# Autodesk Inventor assembly: Assembly1
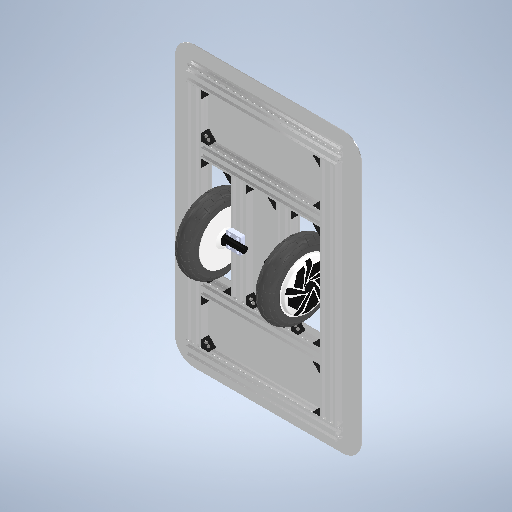
[picture p0: Inventor's stored thumbnail of the model, 512x512]
Saved by Autodesk Inventor 2025 (Build 290162000, 162)
## iProperties
Created: 2025-09-29
Part Number: Assembly1
Document SubType Name: Weldment
Designer: hp
Mass: 4352.41 g
Surface Area: 16168.4 cm^2
Volume: 1611.69 cm^3
Density: 2.70052 g/cm^3
Weld Material: Aluminum 6061, Welded
Author: hp
## Documents named in this file (16)
- D:\gp amr\Assembly1.iam
- D:\gp amr\aluminum-extrusion-beams-1.snapshot.4\2040 - V-Slot\2040 - V-Slot.ipt
- D:\gp amr\corner-brackets-2.snapshot.2\OB-Bracket 2020\OB-Bracket 2020.ipt
- D:\gp amr\nut-m4-2020-10-6mm-1.snapshot.6\2040 - V-Slot.ipt 60.ipt
- D:\gp amr\aluminum-extrusion-beams-1.snapshot.4\2040 - V-Slot\2040 - V-Slot.ipt 320.ipt
- D:\gp amr\plate2mm.ipt
- D:\gp amr\hoverboard-wheel-8-bldc-motor-1.snapshot.4\Motor, BLDC, Hoverboard Wheel, 8.0in\Motor, BLDC, Hoverboard Wheel, 8.0in.ipt
- D:\gp amr\aluminum-extrusion-beams-1.snapshot.4\2040 - V-Slot\2040 - V-Slot.ipt 280.ipt
- D:\gp amr\hoverboard-motor-shaft-retention-bracket-1.snapshot.6\Hub Motor Shaft Bracket\Hub Motor Shaft Bracket.ipt
- D:\t-nut-m5-2020s-1.snapshot.4\T NUT M5 2020S.ipt
- C:\Users\hp\OneDrive - Faculty of Engineering Ain Shams University\Documents\Inventor\Content Center Files\R2025\en-US\ISO 4762(2)\ISO 4762 - M4 x 8ISO.ipt
- D:\gp amr\Assembly1\AIP\FEA\f78c4d0io.fins
- D:\gp amr\Assembly1\AIP\FEA\f78c4d0io.fsat
- D:\gp amr\Assembly1\AIP\FEA\f78c4d0io.ftes
- D:\gp amr\Assembly1\AIP\FEA\f78c4d0io.fwiz
- D:\gp amr\Assembly1\AIP\FEA\f78c4d0ow.fmsh
## Components (114 placed, 10 different names)
1. 2040 - V-Slot:1 — Mate:4, Flush:2, Mate:7, Mate:8, Flush:3, Mate:9, Flush:4, Mate:15, Angle:5, Flush:20, Mate:42, Angle:7, Angle:8
2. 2040 - V-Slot:4 — Mate:11, Mate:12, Flush:5, Mate:17, Mate:19, Mate:21, Angle:11, Angle:12
3. OB-Bracket 2020:1 — Mate:4, Flush:2, Mate:41, Insert:1, Insert:3, Insert:46, Insert:49
4. OB-Bracket 2020:2 — Mate:15, Mate:16, Flush:8, Insert:2, Insert:4, Insert:47, Insert:48
5. OB-Bracket 2020:3 — Mate:19, Mate:20, Flush:10, Insert:7, Insert:8, Insert:54, Insert:55
6. OB-Bracket 2020:4 — Mate:31, Mate:32, Flush:15, Insert:26, Insert:27, Insert:66, Insert:67
7. OB-Bracket 2020:5 — Mate:17, Mate:18, Flush:9, Insert:5, Insert:6, Insert:56, Insert:57
8. OB-Bracket 2020:6 — Mate:23, Mate:24, Flush:11, Insert:28, Insert:29, Insert:72, Insert:73
9. OB-Bracket 2020:7 — Mate:25, Mate:26, Flush:12, Insert:18, Insert:19, Insert:50, Insert:51
10. 2040 - V-Slot.ipt 60:1 — Mate:7, Mate:8, Flush:3, Mate:13, Angle:2, Flush:6, Mate:14, Angle:3, Flush:7, Mate:18, Flush:9, Mate:28, Flush:13, Mate:30, Flush:14, Mate:36, Mate:37, Mate:41, Mate:44, Angle:10, Angle:15, Angle:21, Angle:23
11. 2040 - V-Slot.ipt 60:2 — Mate:9, Flush:4, Mate:11, Mate:12, Flush:5, Mate:16, Flush:8, Mate:20, Flush:10, Mate:24, Mate:26, Mate:32, Flush:15, Mate:34, Flush:16, Mate:39, Angle:4, Flush:19, Mate:40, Mate:47, Angle:9, Angle:17, Angle:18, Angle:25
12. 2040 - V-Slot.ipt 320:1 — Mate:13, Angle:2, Flush:6, Mate:22, Mate:25, Flush:12, Mate:29, Mate:31, Mate:35, Flush:17, Mate:39, Mate:42, Mate:45, Mate:48, Mate:56, Mate:57, Angle:14, Angle:16, Angle:22, Angle:24, Mate:68, Mate:70, Mate:73, Mate:75, Angle:34, Angle:37, Angle:39, Angle:40
13. 2040 - V-Slot.ipt 320:2 — Mate:14, Angle:3, Flush:7, Mate:21, Mate:22, Mate:23, Flush:11, Mate:27, Mate:33, Mate:38, Flush:18, Angle:13, Angle:19, Angle:20, Mate:65, Flush:25, Mate:67, Flush:26, Mate:77, Flush:32, Mate:79, Angle:26, Angle:28, Angle:31, Angle:33, Insert:76
14. OB-Bracket 2020:8 — Mate:27, Mate:28, Flush:13, Insert:22, Insert:23, Insert:74, Insert:75
15. OB-Bracket 2020:9 — Mate:29, Mate:30, Flush:14, Insert:20, Insert:21, Insert:52, Insert:53
16. OB-Bracket 2020:10 — Mate:33, Mate:34, Flush:16, Insert:16, Insert:17, Insert:58, Insert:59
17. OB-Bracket 2020:11 — Mate:35, Mate:36, Flush:17, Insert:24, Insert:25, Insert:83, Insert:84
18. OB-Bracket 2020:12 — Mate:37, Mate:38, Flush:18, Insert:14, Insert:15, Insert:60, Insert:61
19. plate2mm:1 — Angle:4, Angle:5, Flush:19, Mate:40, Flush:20, Flush:21, Flush:22, Mate:43, Mate:46
20. Motor, BLDC, Hoverboard Wheel, 8.0in:1 — Mate:61, Mate:62, Mate:63
21. Motor, BLDC, Hoverboard Wheel, 8.0in:2 — Mate:58, Mate:59, Mate:60
22. 2040 - V-Slot.ipt 280:1 — Mate:43, Mate:44, Mate:45, Mate:55, Flush:24, Mate:66, Mate:69, Flush:28, Mate:74, Flush:31, Mate:78, Flush:33, Angle:27, Angle:30, Angle:36, Angle:41
23. 2040 - V-Slot.ipt 280:2 — Mate:46, Mate:47, Mate:48, Mate:54, Flush:23, Mate:64, Mate:71, Flush:29, Mate:72, Flush:30, Mate:76, Angle:29, Angle:32, Angle:35, Angle:38
24. Hub Motor Shaft Bracket:1 — Mate:54, Mate:56, Flush:23, Mate:61, Mate:62, Mate:63
25. Hub Motor Shaft Bracket:2 — Mate:55, Mate:57, Flush:24, Mate:58, Mate:59, Mate:60
26. T NUT M5 2020S:1 — Insert:2, Angle:8
27. T NUT M5 2020S:2 — Insert:3, Angle:10
28. T NUT M5 2020S:3 — Angle:9, Insert:4
29. T NUT M5 2020S:4 — Insert:1, Angle:7
30. T NUT M5 2020S:5 — Insert:8
31. T NUT M5 2020S:6 — Insert:6, Angle:11
32. T NUT M5 2020S:7 — Insert:7, Angle:12
33. T NUT M5 2020S:8 — Insert:5
34. T NUT M5 2020S:9 — Insert:14
35. T NUT M5 2020S:10 — Insert:15
36. T NUT M5 2020S:11 — Insert:17, Angle:13
37. T NUT M5 2020S:12 — Insert:16
38. T NUT M5 2020S:13 — Insert:18, Angle:17
39. T NUT M5 2020S:14 — Insert:20, Angle:15
40. T NUT M5 2020S:15 — Insert:21, Angle:14
41. T NUT M5 2020S:16 — Insert:19, Angle:16
42. T NUT M5 2020S:17 — Insert:23, Angle:20
43. T NUT M5 2020S:18 — Insert:25, Angle:22
44. T NUT M5 2020S:19 — Insert:26, Angle:24
45. T NUT M5 2020S:20 — Insert:22, Angle:21
46. T NUT M5 2020S:21 — Insert:24, Angle:23
47. T NUT M5 2020S:22 — Insert:27, Angle:25
48. T NUT M5 2020S:23 — Insert:29, Angle:18
49. T NUT M5 2020S:24 — Insert:28, Angle:19
50. OB-Bracket 2020:13 — Mate:74, Mate:75, Flush:31, Insert:30, Insert:31, Insert:79, Insert:80
51. OB-Bracket 2020:14 — Mate:76, Mate:77, Flush:32, Insert:40, Insert:41, Insert:85, Insert:86
52. OB-Bracket 2020:15 — Mate:66, Mate:67, Flush:26, Insert:44, Insert:45, Insert:68, Insert:69
53. OB-Bracket 2020:16 — Mate:68, Mate:69, Flush:28, Insert:36, Insert:37, Insert:62, Insert:63
54. OB-Bracket 2020:17 — Mate:70, Mate:71, Flush:29, Insert:34, Insert:35, Insert:64, Insert:65
55. OB-Bracket 2020:18 — Mate:72, Mate:73, Flush:30, Insert:32, Insert:33, Insert:81, Insert:82
56. OB-Bracket 2020:19 — Mate:78, Mate:79, Flush:33, Insert:38, Insert:39, Insert:77, Insert:78
57. OB-Bracket 2020:20 — Mate:64, Mate:65, Flush:25, Insert:42, Insert:43, Insert:70, Insert:71
58. T NUT M5 2020S:25 — Insert:34, Angle:38
59. T NUT M5 2020S:26 — Insert:37, Angle:40
60. T NUT M5 2020S:27 — Insert:32, Angle:35
61. T NUT M5 2020S:28 — Insert:31, Angle:37
62. T NUT M5 2020S:29 — Insert:33, Angle:34
63. T NUT M5 2020S:30 — Insert:35, Angle:39
64. T NUT M5 2020S:31 — Insert:36, Angle:41
65. T NUT M5 2020S:32 — Insert:30, Angle:36
66. T NUT M5 2020S:33 — Insert:40, Angle:32
67. T NUT M5 2020S:34 — Insert:42, Angle:29
68. T NUT M5 2020S:35 — Insert:38, Angle:30
69. T NUT M5 2020S:36 — Insert:39, Angle:31
70. T NUT M5 2020S:37 — Insert:44, Angle:26
71. T NUT M5 2020S:38 — Insert:43, Angle:28
72. T NUT M5 2020S:39 — Insert:45, Angle:27
73. T NUT M5 2020S:40 — Insert:41, Angle:33
74. ISO 4762 M4 x 8:1 — Insert:46
75. ISO 4762 M4 x 8:2 — Insert:48
76. ISO 4762 M4 x 8:3 — Insert:51
77. ISO 4762 M4 x 8:4 — Insert:52
78. ISO 4762 M4 x 8:5 — Insert:53
79. ISO 4762 M4 x 8:6 — Insert:54
80. ISO 4762 M4 x 8:7 — Insert:55
81. ISO 4762 M4 x 8:8 — Insert:56
82. ISO 4762 M4 x 8:9 — Insert:57
83. ISO 4762 M4 x 8:10 — Insert:58
84. ISO 4762 M4 x 8:11 — Insert:61
85. ISO 4762 M4 x 8:12 — Insert:60
86. ISO 4762 M4 x 8:13 — Insert:59
87. ISO 4762 M4 x 8:14 — Insert:50
88. ISO 4762 M4 x 8:15 — Insert:49
89. ISO 4762 M4 x 8:16 — Insert:47
90. ISO 4762 M4 x 8:17 — Insert:72
91. ISO 4762 M4 x 8:18 — Insert:70
92. ISO 4762 M4 x 8:19 — Insert:71
93. ISO 4762 M4 x 8:20 — Insert:73
94. ISO 4762 M4 x 8:21 — Insert:69
95. ISO 4762 M4 x 8:22 — Insert:67
96. ISO 4762 M4 x 8:23 — Insert:74
97. ISO 4762 M4 x 8:24 — Insert:68
98. ISO 4762 M4 x 8:25 — Insert:62
99. ISO 4762 M4 x 8:26 — Insert:64
100. ISO 4762 M4 x 8:27 — Insert:75
101. ISO 4762 M4 x 8:28 — Insert:66
102. ISO 4762 M4 x 8:29 — Insert:77
103. ISO 4762 M4 x 8:30 — Insert:76
104. ISO 4762 M4 x 8:31 — Insert:65
105. ISO 4762 M4 x 8:32 — Insert:63
106. ISO 4762 M4 x 8:33 — Insert:80
107. ISO 4762 M4 x 8:34 — Insert:84
108. ISO 4762 M4 x 8:35 — Insert:83
109. ISO 4762 M4 x 8:36 — Insert:82
110. ISO 4762 M4 x 8:37 — Insert:81
111. ISO 4762 M4 x 8:38 — Insert:79
112. ISO 4762 M4 x 8:39 — Insert:78
113. ISO 4762 M4 x 8:40 — Insert:85
114. ISO 4762 M4 x 8:43 — Insert:86
## Relationships (219: Insert 81, Mate 68, Angle 39, Flush 31)
- Mate:4: 2040 - V-Slot:1 ↔ OB-Bracket 2020:1
- Flush:2: 2040 - V-Slot:1 ↔ OB-Bracket 2020:1
- Mate:7: 2040 - V-Slot:1 ↔ 2040 - V-Slot.ipt 60:1
- Mate:8: 2040 - V-Slot:1 ↔ 2040 - V-Slot.ipt 60:1
- Flush:3: 2040 - V-Slot:1 ↔ 2040 - V-Slot.ipt 60:1
- Mate:9: 2040 - V-Slot:1 ↔ 2040 - V-Slot.ipt 60:2
- Flush:4: 2040 - V-Slot:1 ↔ 2040 - V-Slot.ipt 60:2
- Mate:11: 2040 - V-Slot:4 ↔ 2040 - V-Slot.ipt 60:2
- Mate:12: 2040 - V-Slot:4 ↔ 2040 - V-Slot.ipt 60:2
- Flush:5: 2040 - V-Slot:4 ↔ 2040 - V-Slot.ipt 60:2
- Mate:13: 2040 - V-Slot.ipt 60:1 ↔ 2040 - V-Slot.ipt 320:1
- Angle:2 (0 deg): 2040 - V-Slot.ipt 60:1 ↔ 2040 - V-Slot.ipt 320:1
- Flush:6: 2040 - V-Slot.ipt 60:1 ↔ 2040 - V-Slot.ipt 320:1
- Mate:14: 2040 - V-Slot.ipt 60:1 ↔ 2040 - V-Slot.ipt 320:2
- Angle:3 (0 deg): 2040 - V-Slot.ipt 60:1 ↔ 2040 - V-Slot.ipt 320:2
- Flush:7: 2040 - V-Slot.ipt 60:1 ↔ 2040 - V-Slot.ipt 320:2
- Mate:15: 2040 - V-Slot:1 ↔ OB-Bracket 2020:2
- Mate:16: OB-Bracket 2020:2 ↔ 2040 - V-Slot.ipt 60:2
- Flush:8: OB-Bracket 2020:2 ↔ 2040 - V-Slot.ipt 60:2
- Mate:17: 2040 - V-Slot:4 ↔ OB-Bracket 2020:5
- Mate:18: OB-Bracket 2020:5 ↔ 2040 - V-Slot.ipt 60:1
- Flush:9: OB-Bracket 2020:5 ↔ 2040 - V-Slot.ipt 60:1
- Mate:19: 2040 - V-Slot:4 ↔ OB-Bracket 2020:3
- Mate:20: OB-Bracket 2020:3 ↔ 2040 - V-Slot.ipt 60:2
- Flush:10: OB-Bracket 2020:3 ↔ 2040 - V-Slot.ipt 60:2
- Mate:21 (120 mm): 2040 - V-Slot:4 ↔ 2040 - V-Slot.ipt 320:2
- Mate:22 (280 mm): 2040 - V-Slot.ipt 320:1 ↔ 2040 - V-Slot.ipt 320:2
- Mate:23: OB-Bracket 2020:6 ↔ 2040 - V-Slot.ipt 320:2
- Mate:24: OB-Bracket 2020:6 ↔ 2040 - V-Slot.ipt 60:2
- Flush:11: OB-Bracket 2020:6 ↔ 2040 - V-Slot.ipt 320:2
- Mate:25: OB-Bracket 2020:7 ↔ 2040 - V-Slot.ipt 320:1
- Mate:26: OB-Bracket 2020:7 ↔ 2040 - V-Slot.ipt 60:2
- Flush:12: OB-Bracket 2020:7 ↔ 2040 - V-Slot.ipt 320:1
- Mate:27: 2040 - V-Slot.ipt 320:2 ↔ OB-Bracket 2020:8
- Mate:28: 2040 - V-Slot.ipt 60:1 ↔ OB-Bracket 2020:8
- Flush:13: 2040 - V-Slot.ipt 60:1 ↔ OB-Bracket 2020:8
- Mate:29: 2040 - V-Slot.ipt 320:1 ↔ OB-Bracket 2020:9
- Mate:30: 2040 - V-Slot.ipt 60:1 ↔ OB-Bracket 2020:9
- Flush:14: 2040 - V-Slot.ipt 60:1 ↔ OB-Bracket 2020:9
- Mate:31: OB-Bracket 2020:4 ↔ 2040 - V-Slot.ipt 320:1
- Mate:32: OB-Bracket 2020:4 ↔ 2040 - V-Slot.ipt 60:2
- Flush:15: OB-Bracket 2020:4 ↔ 2040 - V-Slot.ipt 60:2
- Mate:33: 2040 - V-Slot.ipt 320:2 ↔ OB-Bracket 2020:10
- Mate:34: 2040 - V-Slot.ipt 60:2 ↔ OB-Bracket 2020:10
- Flush:16: 2040 - V-Slot.ipt 60:2 ↔ OB-Bracket 2020:10
- Mate:35: 2040 - V-Slot.ipt 320:1 ↔ OB-Bracket 2020:11
- Mate:36: 2040 - V-Slot.ipt 60:1 ↔ OB-Bracket 2020:11
- Flush:17: 2040 - V-Slot.ipt 320:1 ↔ OB-Bracket 2020:11
- Mate:37: 2040 - V-Slot.ipt 60:1 ↔ OB-Bracket 2020:12
- Mate:38: 2040 - V-Slot.ipt 320:2 ↔ OB-Bracket 2020:12
- Flush:18: 2040 - V-Slot.ipt 320:2 ↔ OB-Bracket 2020:12
- Mate:39: 2040 - V-Slot.ipt 60:2 ↔ 2040 - V-Slot.ipt 320:1
- Angle:4 (0 deg): 2040 - V-Slot.ipt 60:2 ↔ plate2mm:1
- Angle:5 (0 deg): 2040 - V-Slot:1 ↔ plate2mm:1
- Flush:19 (-50 mm): 2040 - V-Slot.ipt 60:2 ↔ plate2mm:1
- Mate:40: 2040 - V-Slot.ipt 60:2 ↔ plate2mm:1
- Flush:20 (35 mm): 2040 - V-Slot:1 ↔ plate2mm:1
- Mate:41: OB-Bracket 2020:1 ↔ 2040 - V-Slot.ipt 60:1
- Flush:21: plate2mm:1
- Flush:22: plate2mm:1
- Mate:42 (120 mm): 2040 - V-Slot:1 ↔ 2040 - V-Slot.ipt 320:1
- Mate:43: plate2mm:1 ↔ 2040 - V-Slot.ipt 280:1
- Mate:44 (80 mm): 2040 - V-Slot.ipt 60:1 ↔ 2040 - V-Slot.ipt 280:1
- Mate:45: 2040 - V-Slot.ipt 320:1 ↔ 2040 - V-Slot.ipt 280:1
- Mate:46: plate2mm:1 ↔ 2040 - V-Slot.ipt 280:2
- Mate:47 (80 mm): 2040 - V-Slot.ipt 60:2 ↔ 2040 - V-Slot.ipt 280:2
- Mate:48: 2040 - V-Slot.ipt 320:1 ↔ 2040 - V-Slot.ipt 280:2
- Mate:54: 2040 - V-Slot.ipt 280:2 ↔ Hub Motor Shaft Bracket:1
- Mate:55: 2040 - V-Slot.ipt 280:1 ↔ Hub Motor Shaft Bracket:2
- Mate:56 (118.64 mm): 2040 - V-Slot.ipt 320:1 ↔ Hub Motor Shaft Bracket:1
- Flush:23: 2040 - V-Slot.ipt 280:2 ↔ Hub Motor Shaft Bracket:1
- Mate:57 (118.64 mm): 2040 - V-Slot.ipt 320:1 ↔ Hub Motor Shaft Bracket:2
- Flush:24: 2040 - V-Slot.ipt 280:1 ↔ Hub Motor Shaft Bracket:2
- Mate:58: Motor, BLDC, Hoverboard Wheel, 8.0in:2 ↔ Hub Motor Shaft Bracket:2
- Mate:59: Motor, BLDC, Hoverboard Wheel, 8.0in:2 ↔ Hub Motor Shaft Bracket:2
- Mate:60 (0.585 mm): Motor, BLDC, Hoverboard Wheel, 8.0in:2 ↔ Hub Motor Shaft Bracket:2
- Mate:61: Motor, BLDC, Hoverboard Wheel, 8.0in:1 ↔ Hub Motor Shaft Bracket:1
- Mate:62: Motor, BLDC, Hoverboard Wheel, 8.0in:1 ↔ Hub Motor Shaft Bracket:1
- Mate:63 (0.585 mm): Motor, BLDC, Hoverboard Wheel, 8.0in:1 ↔ Hub Motor Shaft Bracket:1
- Insert:1 (-0.45 mm): OB-Bracket 2020:1 ↔ T NUT M5 2020S:4
- Angle:7 (0 deg): 2040 - V-Slot:1 ↔ T NUT M5 2020S:4
- Insert:2 (-0.45 mm): OB-Bracket 2020:2 ↔ T NUT M5 2020S:1
- Angle:8 (0 deg): 2040 - V-Slot:1 ↔ T NUT M5 2020S:1
- Insert:3 (-0.45 mm): OB-Bracket 2020:1 ↔ T NUT M5 2020S:2
- Angle:9 (0 deg): 2040 - V-Slot.ipt 60:2 ↔ T NUT M5 2020S:3
- Insert:4 (-0.45 mm): OB-Bracket 2020:2 ↔ T NUT M5 2020S:3
- Angle:10 (0 deg): 2040 - V-Slot.ipt 60:1 ↔ T NUT M5 2020S:2
- Insert:5 (-0.45 mm): OB-Bracket 2020:5 ↔ T NUT M5 2020S:8
- Insert:6 (-0.45 mm): OB-Bracket 2020:5 ↔ T NUT M5 2020S:6
- Angle:11 (0 deg): 2040 - V-Slot:4 ↔ T NUT M5 2020S:6
- Insert:7 (-0.45 mm): OB-Bracket 2020:3 ↔ T NUT M5 2020S:7
- Insert:8 (-0.45 mm): OB-Bracket 2020:3 ↔ T NUT M5 2020S:5
- Angle:12 (0 deg): 2040 - V-Slot:4 ↔ T NUT M5 2020S:7
- Insert:14 (-0.45 mm): OB-Bracket 2020:12 ↔ T NUT M5 2020S:9
- Insert:15 (-0.45 mm): OB-Bracket 2020:12 ↔ T NUT M5 2020S:10
- Insert:16 (0.45 mm): OB-Bracket 2020:10 ↔ T NUT M5 2020S:12
- Insert:17 (0.45 mm): OB-Bracket 2020:10 ↔ T NUT M5 2020S:11
- Angle:13 (0 deg): 2040 - V-Slot.ipt 320:2 ↔ T NUT M5 2020S:11
- Insert:18 (0.45 mm): OB-Bracket 2020:7 ↔ T NUT M5 2020S:13
- Insert:19 (0.45 mm): OB-Bracket 2020:7 ↔ T NUT M5 2020S:16
- Insert:20 (0.45 mm): OB-Bracket 2020:9 ↔ T NUT M5 2020S:14
- Insert:21 (-0.45 mm): OB-Bracket 2020:9 ↔ T NUT M5 2020S:15
- Angle:14 (0 deg): 2040 - V-Slot.ipt 320:1 ↔ T NUT M5 2020S:15
- Angle:15 (0 deg): 2040 - V-Slot.ipt 60:1 ↔ T NUT M5 2020S:14
- Angle:16 (0 deg): 2040 - V-Slot.ipt 320:1 ↔ T NUT M5 2020S:16
- Angle:17 (0 deg): 2040 - V-Slot.ipt 60:2 ↔ T NUT M5 2020S:13
- Insert:22 (0.45 mm): OB-Bracket 2020:8 ↔ T NUT M5 2020S:20
- Insert:23 (0.45 mm): OB-Bracket 2020:8 ↔ T NUT M5 2020S:17
- Insert:24 (-0.45 mm): OB-Bracket 2020:11 ↔ T NUT M5 2020S:21
- Insert:25 (-0.45 mm): OB-Bracket 2020:11 ↔ T NUT M5 2020S:18
- Insert:26 (-0.45 mm): OB-Bracket 2020:4 ↔ T NUT M5 2020S:19
- Insert:27 (-0.45 mm): OB-Bracket 2020:4 ↔ T NUT M5 2020S:22
- Insert:28 (0.45 mm): OB-Bracket 2020:6 ↔ T NUT M5 2020S:24
- Insert:29 (0.45 mm): OB-Bracket 2020:6 ↔ T NUT M5 2020S:23
- Angle:18 (0 deg): 2040 - V-Slot.ipt 60:2 ↔ T NUT M5 2020S:23
- Angle:19 (0 deg): 2040 - V-Slot.ipt 320:2 ↔ T NUT M5 2020S:24
- Angle:20 (0 deg): 2040 - V-Slot.ipt 320:2 ↔ T NUT M5 2020S:17
- Angle:21 (0 deg): 2040 - V-Slot.ipt 60:1 ↔ T NUT M5 2020S:20
- Angle:22 (0 deg): 2040 - V-Slot.ipt 320:1 ↔ T NUT M5 2020S:18
- Angle:23 (0 deg): 2040 - V-Slot.ipt 60:1 ↔ T NUT M5 2020S:21
- Angle:24 (0 deg): 2040 - V-Slot.ipt 320:1 ↔ T NUT M5 2020S:19
- Angle:25 (0 deg): 2040 - V-Slot.ipt 60:2 ↔ T NUT M5 2020S:22
- Mate:64: 2040 - V-Slot.ipt 280:2 ↔ OB-Bracket 2020:20
- Mate:65: 2040 - V-Slot.ipt 320:2 ↔ OB-Bracket 2020:20
- Flush:25: 2040 - V-Slot.ipt 320:2 ↔ OB-Bracket 2020:20
- Mate:66: 2040 - V-Slot.ipt 280:1 ↔ OB-Bracket 2020:15
- Mate:67: 2040 - V-Slot.ipt 320:2 ↔ OB-Bracket 2020:15
- Flush:26: 2040 - V-Slot.ipt 320:2 ↔ OB-Bracket 2020:15
- Mate:68: 2040 - V-Slot.ipt 320:1 ↔ OB-Bracket 2020:16
- Mate:69: 2040 - V-Slot.ipt 280:1 ↔ OB-Bracket 2020:16
- Flush:28: 2040 - V-Slot.ipt 280:1 ↔ OB-Bracket 2020:16
- Mate:70: 2040 - V-Slot.ipt 320:1 ↔ OB-Bracket 2020:17
- Mate:71: 2040 - V-Slot.ipt 280:2 ↔ OB-Bracket 2020:17
- Flush:29: 2040 - V-Slot.ipt 280:2 ↔ OB-Bracket 2020:17
- Mate:72: 2040 - V-Slot.ipt 280:2 ↔ OB-Bracket 2020:18
- Mate:73: 2040 - V-Slot.ipt 320:1 ↔ OB-Bracket 2020:18
- Flush:30: 2040 - V-Slot.ipt 280:2 ↔ OB-Bracket 2020:18
- Mate:74: 2040 - V-Slot.ipt 280:1 ↔ OB-Bracket 2020:13
- Mate:75: 2040 - V-Slot.ipt 320:1 ↔ OB-Bracket 2020:13
- Flush:31: 2040 - V-Slot.ipt 280:1 ↔ OB-Bracket 2020:13
- Mate:76: 2040 - V-Slot.ipt 280:2 ↔ OB-Bracket 2020:14
- Mate:77: 2040 - V-Slot.ipt 320:2 ↔ OB-Bracket 2020:14
- Flush:32: 2040 - V-Slot.ipt 320:2 ↔ OB-Bracket 2020:14
- Mate:78: 2040 - V-Slot.ipt 280:1 ↔ OB-Bracket 2020:19
- Mate:79: 2040 - V-Slot.ipt 320:2 ↔ OB-Bracket 2020:19
- Flush:33: 2040 - V-Slot.ipt 280:1 ↔ OB-Bracket 2020:19
- Insert:30 (0.45 mm): OB-Bracket 2020:13 ↔ T NUT M5 2020S:32
- Insert:31 (0.45 mm): OB-Bracket 2020:13 ↔ T NUT M5 2020S:28
- Insert:32 (0.45 mm): OB-Bracket 2020:18 ↔ T NUT M5 2020S:27
- Insert:33 (0.45 mm): OB-Bracket 2020:18 ↔ T NUT M5 2020S:29
- Insert:34 (0.45 mm): OB-Bracket 2020:17 ↔ T NUT M5 2020S:25
- Insert:35 (0.45 mm): OB-Bracket 2020:17 ↔ T NUT M5 2020S:30
- Insert:36 (0.45 mm): OB-Bracket 2020:16 ↔ T NUT M5 2020S:31
- Insert:37 (0.45 mm): OB-Bracket 2020:16 ↔ T NUT M5 2020S:26
- Insert:38 (0.45 mm): OB-Bracket 2020:19 ↔ T NUT M5 2020S:35
- Insert:39 (0.45 mm): OB-Bracket 2020:19 ↔ T NUT M5 2020S:36
- Insert:40 (0.45 mm): OB-Bracket 2020:14 ↔ T NUT M5 2020S:33
- Insert:41 (0.45 mm): OB-Bracket 2020:14 ↔ T NUT M5 2020S:40
- Insert:42 (0.45 mm): OB-Bracket 2020:20 ↔ T NUT M5 2020S:34
- Insert:43 (0.45 mm): OB-Bracket 2020:20 ↔ T NUT M5 2020S:38
- Insert:44 (0.45 mm): OB-Bracket 2020:15 ↔ T NUT M5 2020S:37
- Insert:45 (0.45 mm): OB-Bracket 2020:15 ↔ T NUT M5 2020S:39
- Angle:26 (0 deg): 2040 - V-Slot.ipt 320:2 ↔ T NUT M5 2020S:37
- Angle:27 (0 deg): 2040 - V-Slot.ipt 280:1 ↔ T NUT M5 2020S:39
- Angle:28 (0 deg): 2040 - V-Slot.ipt 320:2 ↔ T NUT M5 2020S:38
- Angle:29 (0 deg): 2040 - V-Slot.ipt 280:2 ↔ T NUT M5 2020S:34
- Angle:30 (0 deg): 2040 - V-Slot.ipt 280:1 ↔ T NUT M5 2020S:35
- Angle:31 (0 deg): 2040 - V-Slot.ipt 320:2 ↔ T NUT M5 2020S:36
- Angle:32 (0 deg): 2040 - V-Slot.ipt 280:2 ↔ T NUT M5 2020S:33
- Angle:33 (0 deg): 2040 - V-Slot.ipt 320:2 ↔ T NUT M5 2020S:40
- Angle:34 (0 deg): 2040 - V-Slot.ipt 320:1 ↔ T NUT M5 2020S:29
- Angle:35 (0 deg): 2040 - V-Slot.ipt 280:2 ↔ T NUT M5 2020S:27
- Angle:36 (0 deg): 2040 - V-Slot.ipt 280:1 ↔ T NUT M5 2020S:32
- Angle:37 (0 deg): 2040 - V-Slot.ipt 320:1 ↔ T NUT M5 2020S:28
- Angle:38 (0 deg): 2040 - V-Slot.ipt 280:2 ↔ T NUT M5 2020S:25
- Angle:39 (0 deg): 2040 - V-Slot.ipt 320:1 ↔ T NUT M5 2020S:30
- Angle:40 (0 deg): 2040 - V-Slot.ipt 320:1 ↔ T NUT M5 2020S:26
- Angle:41 (0 deg): 2040 - V-Slot.ipt 280:1 ↔ T NUT M5 2020S:31
- Insert:46: OB-Bracket 2020:1 ↔ ISO 4762 M4 x 8:1
- Insert:47: OB-Bracket 2020:2 ↔ ISO 4762 M4 x 8:16
- Insert:48: OB-Bracket 2020:2 ↔ ISO 4762 M4 x 8:2
- Insert:49: OB-Bracket 2020:1 ↔ ISO 4762 M4 x 8:15
- Insert:50: OB-Bracket 2020:7 ↔ ISO 4762 M4 x 8:14
- Insert:51: OB-Bracket 2020:7 ↔ ISO 4762 M4 x 8:3
- Insert:52: OB-Bracket 2020:9 ↔ ISO 4762 M4 x 8:4
- Insert:53: OB-Bracket 2020:9 ↔ ISO 4762 M4 x 8:5
- Insert:54: OB-Bracket 2020:3 ↔ ISO 4762 M4 x 8:6
- Insert:55: OB-Bracket 2020:3 ↔ ISO 4762 M4 x 8:7
- Insert:56: OB-Bracket 2020:5 ↔ ISO 4762 M4 x 8:8
- Insert:57: OB-Bracket 2020:5 ↔ ISO 4762 M4 x 8:9
- Insert:58: OB-Bracket 2020:10 ↔ ISO 4762 M4 x 8:10
- Insert:59: OB-Bracket 2020:10 ↔ ISO 4762 M4 x 8:13
- Insert:60: OB-Bracket 2020:12 ↔ ISO 4762 M4 x 8:12
- Insert:61: OB-Bracket 2020:12 ↔ ISO 4762 M4 x 8:11
- Insert:62: OB-Bracket 2020:16 ↔ ISO 4762 M4 x 8:25
- Insert:63: OB-Bracket 2020:16 ↔ ISO 4762 M4 x 8:32
- Insert:64: OB-Bracket 2020:17 ↔ ISO 4762 M4 x 8:26
- Insert:65: OB-Bracket 2020:17 ↔ ISO 4762 M4 x 8:31
- Insert:66: OB-Bracket 2020:4 ↔ ISO 4762 M4 x 8:28
- Insert:67: OB-Bracket 2020:4 ↔ ISO 4762 M4 x 8:22
- Insert:68: OB-Bracket 2020:15 ↔ ISO 4762 M4 x 8:24
- Insert:69: OB-Bracket 2020:15 ↔ ISO 4762 M4 x 8:21
- Insert:70: OB-Bracket 2020:20 ↔ ISO 4762 M4 x 8:18
- Insert:71: OB-Bracket 2020:20 ↔ ISO 4762 M4 x 8:19
- Insert:72: OB-Bracket 2020:6 ↔ ISO 4762 M4 x 8:17
- Insert:73: OB-Bracket 2020:6 ↔ ISO 4762 M4 x 8:20
- Insert:74: OB-Bracket 2020:8 ↔ ISO 4762 M4 x 8:23
- Insert:75: OB-Bracket 2020:8 ↔ ISO 4762 M4 x 8:27
- Insert:76: 2040 - V-Slot.ipt 320:2 ↔ ISO 4762 M4 x 8:30
- Insert:77: OB-Bracket 2020:19 ↔ ISO 4762 M4 x 8:29
- Insert:78: OB-Bracket 2020:19 ↔ ISO 4762 M4 x 8:39
- Insert:79: OB-Bracket 2020:13 ↔ ISO 4762 M4 x 8:38
- Insert:80: OB-Bracket 2020:13 ↔ ISO 4762 M4 x 8:33
- Insert:81: OB-Bracket 2020:18 ↔ ISO 4762 M4 x 8:37
- Insert:82: OB-Bracket 2020:18 ↔ ISO 4762 M4 x 8:36
- Insert:83: OB-Bracket 2020:11 ↔ ISO 4762 M4 x 8:35
- Insert:84: OB-Bracket 2020:11 ↔ ISO 4762 M4 x 8:34
- Insert:85: OB-Bracket 2020:14 ↔ ISO 4762 M4 x 8:40
- Insert:86: OB-Bracket 2020:14 ↔ ISO 4762 M4 x 8:43
## Named parameters: sa_0 = 100000
note: some values were not read from the file. Shown as the stored number, unit unknown: "sa_0".
